# Autodesk Inventor assembly: base_wall_added_MIR
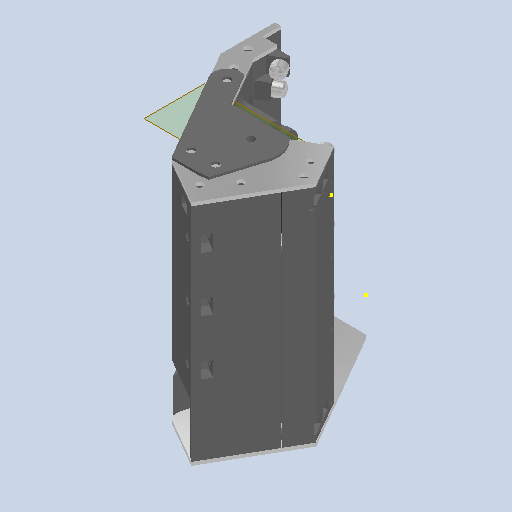
[picture p0: Inventor's stored thumbnail of the model, 512x512]
Saved by Autodesk Inventor 2024.1 (Build 281209000, 209)
## iProperties
Created: 2025-01-18
Part Number: base_wall_added_MIR
Document SubType Name: Assembly
Designer: hibik
Author: hibik
## Documents named in this file (5)
- C:\Users\hibik\Documents\Robomech\RESCUE\ORCA\hard\fork\right\base_wall_added_MIR.iam
- C:\Users\hibik\Documents\Robomech\RESCUE\ORCA\hard\fork\right\base_MIR.iam
- C:\Users\hibik\Documents\Robomech\RESCUE\ORCA\hard\fork\right\base_backwall_setter_upper_MIR.ipt
- C:\Users\hibik\Documents\Robomech\RESCUE\ORCA\hard\fork\right\chain_base_connector_MIR.ipt
- C:\Users\hibik\Documents\Robomech\RESCUE\ORCA\hard\fork\right\screw_cover_upper_MIR.ipt
## Components (4 placed, 4 different names)
1. base_MIR:1 [sub-assembly] — フラッシュ:2, フラッシュ:1, メイト:1, フラッシュ:4, フラッシュ:3, メイト:2, 角度:1, 挿入:1
2. base_backwall_setter_upper_MIR:1 — フラッシュ:2, フラッシュ:1, メイト:1
3. chain_base_connector_MIR:1 — フラッシュ:4, フラッシュ:3, メイト:2
4. screw_cover_upper_MIR:1 — 角度:1, 挿入:1
## Relationships (8: Flush 4, Mate 2, Angle 1, Insert 1)
- フラッシュ:2 [Flush]: base_MIR:1 ↔ base_backwall_setter_upper_MIR:1
- フラッシュ:1 [Flush]: base_MIR:1 ↔ base_backwall_setter_upper_MIR:1
- メイト:1 [Mate]: base_MIR:1 ↔ base_backwall_setter_upper_MIR:1
- フラッシュ:4 [Flush]: base_MIR:1 ↔ chain_base_connector_MIR:1
- フラッシュ:3 [Flush]: base_MIR:1 ↔ chain_base_connector_MIR:1
- メイト:2 [Mate]: base_MIR:1 ↔ chain_base_connector_MIR:1
- 角度:1 [Angle] (180 deg): base_MIR:1 ↔ screw_cover_upper_MIR:1
- 挿入:1 [Insert]: base_MIR:1 ↔ screw_cover_upper_MIR:1
